# Autodesk Inventor assembly: SAR330
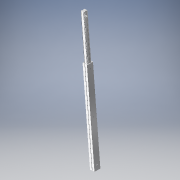
[picture p0: Inventor's stored thumbnail of the model, 180x180]
Saved by Autodesk Inventor 2019 (Build 230136000, 136)
## iProperties
Category: PARTsolutions
Company: MISUMI
Created: 2019-04-19
Part Number: SAR330
Catalog Web Link: www.cadenas.de
Description: SAR3-Slide Rails - Aluminum Alloy - Three-Step Slide Rails
Vendor: MISUMI
Document SubType Name: Assembly
Designer: psadmin
Manufacturer: MISUMI
Mass: 180.874 g
Surface Area: 598.523 cm^2
Volume: 66.9905 cm^3
Density: 2.7 g/cm^3
Title: SAR330
Author: Cadenas PARTsolutions
Comments: Slide Rails - Aluminum Alloy - Three-Step Slide Rails
## Documents named in this file (4)
- C:\Robotics\CAD\COTSParts\Misumi_Slides\AIS2018\SAR330.iam
- C:\Robotics\CAD\COTSParts\Misumi_Slides\AIS2018\SAR330-30_r.ipt
- C:\Robotics\CAD\COTSParts\Misumi_Slides\AIS2018\SAR330-30_b.ipt
- C:\Robotics\CAD\COTSParts\Misumi_Slides\AIS2018\SAR330_ba.ipt
## Components (7 placed, 3 different names)
1. SAR330-30_r:1 — Tangent:1, Tangent:2, Tangent:3, Tangent:4, Tangent:5, Tangent:6, Tangent:7, Tangent:8, Tangent:16, Tangent:17, Tangent:18, Tangent:19, Tangent:20, Tangent:21, Tangent:22, Tangent:23, Flush:2
2. SAR330-30_b:1 — Tangent:9, Tangent:11, Tangent:15, Tangent:24, Tangent:25, Tangent:29, Tangent:31, Flush:1, Flush:2
3. SAR330-30_b:2 — Tangent:10, Tangent:12, Tangent:13, Tangent:14, Tangent:26, Tangent:27, Tangent:28, Tangent:30, Flush:1
4. SAR330_ba:1 — Tangent:4, Tangent:8, Tangent:12, Tangent:14, Tangent:20, Tangent:21, Tangent:27, Tangent:30
5. SAR330_ba:2 — Tangent:1, Tangent:6, Tangent:10, Tangent:13, Tangent:16, Tangent:17, Tangent:26, Tangent:28
6. SAR330_ba:3 — Tangent:2, Tangent:5, Tangent:9, Tangent:18, Tangent:19, Tangent:24, Tangent:29
7. SAR330_ba:4 — Tangent:3, Tangent:7, Tangent:11, Tangent:15, Tangent:22, Tangent:23, Tangent:25, Tangent:31
## Relationships (33: Tangent 31, Flush 2)
- Tangent:1: SAR330-30_r:1 ↔ SAR330_ba:2
- Tangent:2: SAR330-30_r:1 ↔ SAR330_ba:3
- Tangent:3: SAR330-30_r:1 ↔ SAR330_ba:4
- Tangent:4: SAR330-30_r:1 ↔ SAR330_ba:1
- Tangent:5: SAR330-30_r:1 ↔ SAR330_ba:3
- Tangent:6: SAR330-30_r:1 ↔ SAR330_ba:2
- Tangent:7: SAR330-30_r:1 ↔ SAR330_ba:4
- Tangent:8: SAR330-30_r:1 ↔ SAR330_ba:1
- Tangent:9: SAR330-30_b:1 ↔ SAR330_ba:3
- Tangent:10: SAR330-30_b:2 ↔ SAR330_ba:2
- Tangent:11: SAR330-30_b:1 ↔ SAR330_ba:4
- Tangent:12: SAR330-30_b:2 ↔ SAR330_ba:1
- Tangent:13: SAR330-30_b:2 ↔ SAR330_ba:2
- Tangent:14: SAR330-30_b:2 ↔ SAR330_ba:1
- Tangent:15: SAR330-30_b:1 ↔ SAR330_ba:4
- Tangent:16: SAR330-30_r:1 ↔ SAR330_ba:2
- Tangent:17: SAR330-30_r:1 ↔ SAR330_ba:2
- Tangent:18: SAR330-30_r:1 ↔ SAR330_ba:3
- Tangent:19: SAR330-30_r:1 ↔ SAR330_ba:3
- Tangent:20: SAR330-30_r:1 ↔ SAR330_ba:1
- Tangent:21: SAR330-30_r:1 ↔ SAR330_ba:1
- Tangent:22: SAR330-30_r:1 ↔ SAR330_ba:4
- Tangent:23: SAR330-30_r:1 ↔ SAR330_ba:4
- Tangent:24: SAR330-30_b:1 ↔ SAR330_ba:3
- Tangent:25: SAR330-30_b:1 ↔ SAR330_ba:4
- Tangent:26: SAR330-30_b:2 ↔ SAR330_ba:2
- Tangent:27: SAR330-30_b:2 ↔ SAR330_ba:1
- Tangent:28: SAR330-30_b:2 ↔ SAR330_ba:2
- Tangent:29: SAR330-30_b:1 ↔ SAR330_ba:3
- Tangent:30: SAR330-30_b:2 ↔ SAR330_ba:1
- Tangent:31: SAR330-30_b:1 ↔ SAR330_ba:4
- Flush:1: SAR330-30_b:1 ↔ SAR330-30_b:2
- Flush:2: SAR330-30_r:1 ↔ SAR330-30_b:1
